# Autodesk Inventor assembly: Ensamble
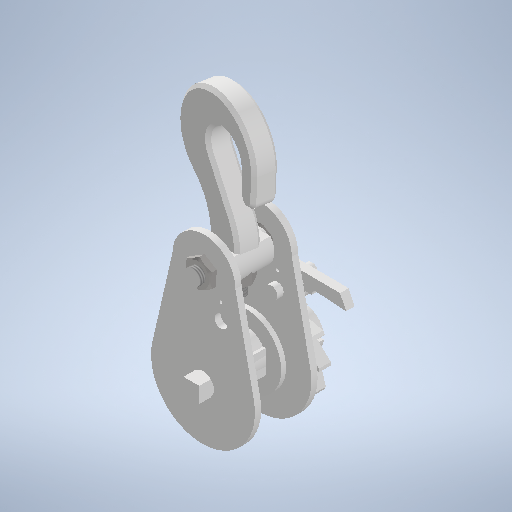
[picture p0: Inventor's stored thumbnail of the model, 512x512]
Saved by Autodesk Inventor 2025.3 (Build 293356030, 356C)
## iProperties
Created: 2025-08-24
Part Number: Ensamble
Document SubType Name: Assembly
Designer: PC
Author: PC
## Documents named in this file (14)
- C:\Users\PC\Desktop\Proyecto emsamble DMW IIQ\Ensamble.iam
- C:\Users\PC\Desktop\Proyecto emsamble DMW IIQ\Cubierta de acoplamiento(pieza 2).ipt
- C:\Users\PC\Desktop\Proyecto emsamble DMW IIQ\Gancho(pieza 6).ipt
- C:\Users\PC\Desktop\Proyecto emsamble DMW IIQ\Pieza 3.ipt
- C:\Users\PC\Desktop\Proyecto emsamble DMW IIQ\Pieza 4.ipt
- C:\Users\PC\Desktop\Proyecto emsamble DMW IIQ\Pieza 5.ipt
- C:\Users\PC\Desktop\Proyecto emsamble DMW IIQ\Pieza 7.ipt
- C:\Users\PC\Desktop\Proyecto emsamble DMW IIQ\Pieza 8.ipt
- C:\Users\PC\Desktop\Proyecto emsamble DMW IIQ\Pieza 9.ipt
- C:\Users\PC\Desktop\Proyecto emsamble DMW IIQ\Pieza 10.ipt
- C:\Users\PC\Desktop\Proyecto emsamble DMW IIQ\Pieza 11.ipt
- C:\Users\PC\Desktop\Proyecto emsamble DMW IIQ\Placa de soporte(pieza 1).ipt
- C:\Users\PC\Documents\Inventor\Content Center Files\R2025\en-US\ISO 4032(2)\ISO 4032 - M12 - ISO.ipt
- C:\Users\PC\Documents\Inventor\Content Center Files\R2025\en-US\ISO 4032(2)\ISO 4032 - M10 - ISO.ipt
## Components (15 placed, 13 different names)
1. Cubierta de acoplamiento(pieza 2):1 — Insert:6
2. Gancho(pieza 6):1 — Insert:4, Insert:10
3. Pieza 3:1 — Flush:1, Mate:2
4. Pieza 4:1 — Insert:9
5. Pieza 8:1 — Mate:1
6. Pieza 9:1 — Insert:3, Mate:1, Flush:1, Mate:2, Insert:6
7. Pieza 10:1 — Insert:7, Insert:8, Insert:9
8. Pieza 11:1 — Insert:1, Insert:2, Insert:4, Insert:11, Insert:12
9. Placa de soporte(pieza 1):1 — Insert:2, Flush:2
10. Pieza 5:2 — Insert:8
11. Pieza 7:2 — Insert:5
12. Placa de soporte(pieza 1):2 — Insert:1, Insert:3, Insert:5, Insert:7, Flush:2
13. ISO 4032 M12:1 — Insert:10
14. ISO 4032 M10:1 — Insert:11
15. ISO 4032 M10:2 — Insert:12
## Relationships (16: Insert 12, Mate 2, Flush 2)
- Insert:1: Pieza 11:1 ↔ Placa de soporte(pieza 1):2
- Insert:2: Pieza 11:1 ↔ Placa de soporte(pieza 1):1
- Insert:3: Pieza 9:1 ↔ Placa de soporte(pieza 1):2
- Mate:1: Pieza 8:1 ↔ Pieza 9:1
- Insert:4: Gancho(pieza 6):1 ↔ Pieza 11:1
- Insert:5: Pieza 7:2 ↔ Placa de soporte(pieza 1):2
- Flush:1: Pieza 3:1 ↔ Pieza 9:1
- Mate:2: Pieza 3:1 ↔ Pieza 9:1
- Insert:6: Cubierta de acoplamiento(pieza 2):1 ↔ Pieza 9:1
- Insert:7: Pieza 10:1 ↔ Placa de soporte(pieza 1):2
- Insert:8: Pieza 10:1 ↔ Pieza 5:2
- Insert:9: Pieza 4:1 ↔ Pieza 10:1
- Flush:2: Placa de soporte(pieza 1):1 ↔ Placa de soporte(pieza 1):2
- Insert:10: Gancho(pieza 6):1 ↔ ISO 4032 M12:1
- Insert:11: Pieza 11:1 ↔ ISO 4032 M10:1
- Insert:12: Pieza 11:1 ↔ ISO 4032 M10:2
